# Autodesk Inventor assembly: Control de produndidad
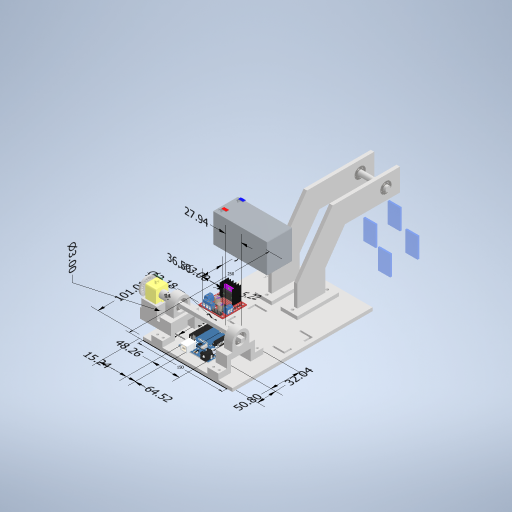
[picture p0: Inventor's stored thumbnail of the model, 512x512]
Saved by Autodesk Inventor 2023 (Build 270158000, 158)
## iProperties
Created: 2023-06-06
Part Number: Control de produndidad
Document SubType Name: Assembly
Designer: sergi
Author: sergi
## Documents named in this file (18)
- C:\Users\sergi\OneDrive\Escritorio\Diseño polea\Control de produndidad.iam
- C:\Users\sergi\OneDrive\Escritorio\Diseño polea\Base.ipt
- C:\Users\sergi\OneDrive\Escritorio\Diseño polea\MotoReductor.ipt
- C:\Users\sergi\OneDrive\Escritorio\Diseño polea\Soporte_motor.ipt
- C:\Users\sergi\OneDrive\Documentos\Inventor\Content Center Files\R2023\es-ES\JIS B 1111(1)\JIS B 1111 - M4,5x20(1).ipt
- C:\Users\sergi\OneDrive\Escritorio\Diseño polea\soporte_balineras.ipt
- C:\Users\sergi\OneDrive\Documentos\Inventor\Content Center Files\R2023\es-ES\DIN 625 - T1\DIN 625 T1 - 619_9 - 9 x 20 x 6.ipt
- C:\Users\sergi\OneDrive\Escritorio\Diseño polea\Adaptador.ipt
- C:\Users\sergi\OneDrive\Escritorio\Diseño polea\barra.ipt
- C:\Users\sergi\OneDrive\Escritorio\Diseño polea\soporte_peso.ipt
- C:\Users\sergi\OneDrive\Escritorio\Diseño polea\Eje.ipt
- C:\Users\sergi\OneDrive\Escritorio\Diseño polea\sotenedor.ipt
- C:\Users\sergi\OneDrive\Escritorio\Diseño polea\Disco_encoder.ipt
- C:\Users\sergi\OneDrive\Escritorio\Diseño polea\FC-03.ipt
- C:\Users\sergi\OneDrive\Escritorio\Diseño polea\Arduino uno R3\arduino uno.ipt
- C:\Users\sergi\OneDrive\Escritorio\Diseño polea\L298N.ipt
- C:\Users\sergi\OneDrive\Escritorio\Diseño polea\Bateria_12v.ipt
- C:\Users\sergi\OneDrive\Escritorio\Diseño polea\base_bateria1.ipt
## Components (27 placed, 17 different names)
1. Base:1 — Coincidencia:1, Coincidencia:2, Nivelación:1, Coincidencia:12, Coincidencia:14, Coincidencia:27, Nivelación:2, Coincidencia:29, Coincidencia:30, Coincidencia:32, Coincidencia:33, Coincidencia:43, Coincidencia:44, Coincidencia:45, Coincidencia:46, Coincidencia:50, Coincidencia:51, Coincidencia:52, Coincidencia:53, Coincidencia:54, Coincidencia:55, Coincidencia:56, Coincidencia:58, Coincidencia:59, Coincidencia:60, Coincidencia:61, Coincidencia:62, Coincidencia:63, Coincidencia:64, Coincidencia:65, Coincidencia:66, Coincidencia:67, Coincidencia:68, Coincidencia:69, Coincidencia:70, Coincidencia:71
2. Soporte_motor:1 — Coincidencia:1, Coincidencia:2, Nivelación:1, Coincidencia:8, Coincidencia:9, Coincidencia:10, Coincidencia:11, Coincidencia:19, Coincidencia:20, Coincidencia:21, Coincidencia:22, Coincidencia:48, Coincidencia:49
3. JIS B 1111 M4,5x20:2 — Coincidencia:8, Coincidencia:9
4. JIS B 1111 M4,5x20:3 — Coincidencia:10, Coincidencia:11
5. soporte_balineras:1 — Coincidencia:12, Coincidencia:14, Coincidencia:16, Coincidencia:17, Coincidencia:19, Coincidencia:52, Coincidencia:53, Coincidencia:54, Coincidencia:55, Coincidencia:56
6. DIN 625 - T1 619/9 - 9 x 20 x 6:1 — Coincidencia:16, Coincidencia:17
7. Adaptador:1 — Coincidencia:23, Coincidencia:24, Coincidencia:25, Coincidencia:26
8. MotoReductor:1 — Coincidencia:20, Coincidencia:21, Coincidencia:22, Coincidencia:23, Coincidencia:24, Coincidencia:47, Nivelación:3, Coincidencia:57
9. barra:2 — Coincidencia:25, Coincidencia:26
10. soporte_balineras:2 — Coincidencia:27, Nivelación:2, Coincidencia:28, Coincidencia:31, Coincidencia:50, Coincidencia:51
11. DIN 625 - T1 619/9 - 9 x 20 x 6:2 — Coincidencia:28, Coincidencia:31
12. soporte_peso:1 — Coincidencia:29, Coincidencia:30, Coincidencia:34, Coincidencia:38
13. soporte_peso:2 — Coincidencia:32, Coincidencia:33, Coincidencia:36, Coincidencia:39
14. DIN 625 - T1 619/9 - 9 x 20 x 6:3 — Coincidencia:34, Coincidencia:38, Coincidencia:41
15. DIN 625 - T1 619/9 - 9 x 20 x 6:4 — Coincidencia:36, Coincidencia:39, Coincidencia:40, Coincidencia:42
16. Eje:1 — Coincidencia:40, Coincidencia:41, Coincidencia:42
17. sotenedor:1 — Coincidencia:45, Coincidencia:46
18. sotenedor:2 — Coincidencia:43, Coincidencia:44
19. Disco_encoder:1 — Coincidencia:47, Nivelación:3, Coincidencia:57
20. FC-03:1 — Coincidencia:48, Coincidencia:49
21. arduino uno:1 — Coincidencia:58, Coincidencia:59, Coincidencia:60, Coincidencia:61, Coincidencia:62, Coincidencia:70
22. L298N:2 — Coincidencia:63, Coincidencia:64, Coincidencia:65, Coincidencia:66, Coincidencia:67, Coincidencia:68, Coincidencia:69, Coincidencia:71
23. Bateria_12v:1
24. base_bateria1:1
25. base_bateria1:2
26. base_bateria1:3
27. base_bateria1:4
## Relationships (64: Mate 61, Flush 3)
- Coincidencia:1 [Mate]: Base:1 ↔ Soporte_motor:1
- Coincidencia:2 [Mate]: Base:1 ↔ Soporte_motor:1
- Nivelación:1 [Flush] (25 mm): Base:1 ↔ Soporte_motor:1
- Coincidencia:8 [Mate]: Soporte_motor:1 ↔ JIS B 1111 M4,5x20:2
- Coincidencia:9 [Mate]: Soporte_motor:1 ↔ JIS B 1111 M4,5x20:2
- Coincidencia:10 [Mate]: Soporte_motor:1 ↔ JIS B 1111 M4,5x20:3
- Coincidencia:11 [Mate]: Soporte_motor:1 ↔ JIS B 1111 M4,5x20:3
- Coincidencia:12 [Mate]: Base:1 ↔ soporte_balineras:1
- Coincidencia:14 [Mate]: Base:1 ↔ soporte_balineras:1
- Coincidencia:16 [Mate]: soporte_balineras:1 ↔ DIN 625 - T1 619/9 - 9 x 20 x 6:1
- Coincidencia:17 [Mate] (-5 mm): soporte_balineras:1 ↔ DIN 625 - T1 619/9 - 9 x 20 x 6:1
- Coincidencia:19 [Mate] (-10 mm): Soporte_motor:1 ↔ soporte_balineras:1
- Coincidencia:20 [Mate]: Soporte_motor:1 ↔ MotoReductor:1
- Coincidencia:21 [Mate] (0.5 mm): Soporte_motor:1 ↔ MotoReductor:1
- Coincidencia:22 [Mate] (0.8 mm): Soporte_motor:1 ↔ MotoReductor:1
- Coincidencia:23 [Mate]: Adaptador:1 ↔ MotoReductor:1
- Coincidencia:24 [Mate]: Adaptador:1 ↔ MotoReductor:1
- Coincidencia:25 [Mate]: Adaptador:1 ↔ barra:2
- Coincidencia:26 [Mate]: Adaptador:1 ↔ barra:2
- Coincidencia:27 [Mate]: Base:1 ↔ soporte_balineras:2
- Nivelación:2 [Flush] (15 mm): Base:1 ↔ soporte_balineras:2
- Coincidencia:28 [Mate]: soporte_balineras:2 ↔ DIN 625 - T1 619/9 - 9 x 20 x 6:2
- Coincidencia:29 [Mate]: Base:1 ↔ soporte_peso:1
- Coincidencia:30 [Mate]: Base:1 ↔ soporte_peso:1
- Coincidencia:31 [Mate] (-10 mm): soporte_balineras:2 ↔ DIN 625 - T1 619/9 - 9 x 20 x 6:2
- Coincidencia:32 [Mate]: Base:1 ↔ soporte_peso:2
- Coincidencia:33 [Mate]: Base:1 ↔ soporte_peso:2
- Coincidencia:34 [Mate]: soporte_peso:1 ↔ DIN 625 - T1 619/9 - 9 x 20 x 6:3
- Coincidencia:36 [Mate]: soporte_peso:2 ↔ DIN 625 - T1 619/9 - 9 x 20 x 6:4
- Coincidencia:38 [Mate] (-6 mm): soporte_peso:1 ↔ DIN 625 - T1 619/9 - 9 x 20 x 6:3
- Coincidencia:39 [Mate] (-6 mm): soporte_peso:2 ↔ DIN 625 - T1 619/9 - 9 x 20 x 6:4
- Coincidencia:40 [Mate]: DIN 625 - T1 619/9 - 9 x 20 x 6:4 ↔ Eje:1
- Coincidencia:41 [Mate]: DIN 625 - T1 619/9 - 9 x 20 x 6:3 ↔ Eje:1
- Coincidencia:42 [Mate] (-4 mm): DIN 625 - T1 619/9 - 9 x 20 x 6:4 ↔ Eje:1
- Coincidencia:43 [Mate]: Base:1 ↔ sotenedor:2
- Coincidencia:44 [Mate]: Base:1 ↔ sotenedor:2
- Coincidencia:45 [Mate]: Base:1 ↔ sotenedor:1
- Coincidencia:46 [Mate]: Base:1 ↔ sotenedor:1
- Coincidencia:47 [Mate]: MotoReductor:1 ↔ Disco_encoder:1
- Nivelación:3 [Flush] (1 mm): MotoReductor:1 ↔ Disco_encoder:1
- Coincidencia:48 [Mate]: Soporte_motor:1 ↔ FC-03:1
- Coincidencia:49 [Mate]: Soporte_motor:1 ↔ FC-03:1
- Coincidencia:50 [Mate]: Base:1 ↔ soporte_balineras:2
- Coincidencia:51 [Mate]: Base:1 ↔ soporte_balineras:2
- Coincidencia:52 [Mate]: Base:1 ↔ soporte_balineras:1
- Coincidencia:53 [Mate]: Base:1 ↔ soporte_balineras:1
- Coincidencia:54 [Mate]: Base:1 ↔ soporte_balineras:1
- Coincidencia:55 [Mate]: Base:1 ↔ soporte_balineras:1
- Coincidencia:56 [Mate]: Base:1 ↔ soporte_balineras:1
- Coincidencia:57 [Mate]: MotoReductor:1 ↔ Disco_encoder:1
- Coincidencia:58 [Mate]: Base:1 ↔ arduino uno:1
- Coincidencia:59 [Mate]: Base:1 ↔ arduino uno:1
- Coincidencia:60 [Mate]: Base:1 ↔ arduino uno:1
- Coincidencia:61 [Mate]: Base:1 ↔ arduino uno:1
- Coincidencia:62 [Mate]: Base:1 ↔ arduino uno:1
- Coincidencia:63 [Mate]: Base:1 ↔ L298N:2
- Coincidencia:64 [Mate]: Base:1 ↔ L298N:2
- Coincidencia:65 [Mate]: Base:1 ↔ L298N:2
- Coincidencia:66 [Mate]: Base:1 ↔ L298N:2
- Coincidencia:67 [Mate]: Base:1 ↔ L298N:2
- Coincidencia:68 [Mate]: Base:1 ↔ L298N:2
- Coincidencia:69 [Mate]: Base:1 ↔ L298N:2
- Coincidencia:70 [Mate]: Base:1 ↔ arduino uno:1
- Coincidencia:71 [Mate]: Base:1 ↔ L298N:2
